# Autodesk Inventor assembly: GCS_AX1
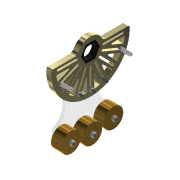
[picture p0: Inventor's stored thumbnail of the model, 180x180]
Saved by Autodesk Inventor 2022 (Build 260153000, 153)
## iProperties
Created: 2022-12-23
Part Number: GCS_AX1
Document SubType Name: Assembly
Designer: alexw
Author: alexw
## Documents named in this file (9)
- C:\Users\alexw\Documents\Inventor\Projects\03_CurrentProjects\MasterThesis\PSM_V1_Rillenkugellager\GCS_AX1.iam
- C:\Users\alexw\Documents\Inventor\Projects\03_CurrentProjects\MasterThesis\PSM_V1_Rillenkugellager\Capstonradialdisc_v2.ipt
- C:\Users\alexw\Documents\Inventor\Projects\03_CurrentProjects\MasterThesis\PSM_V1_Rillenkugellager\CapstonCounterweight_assembly.iam
- C:\Users\alexw\Documents\Inventor\Projects\03_CurrentProjects\MasterThesis\PSM_V1_Rillenkugellager\ContentCenter\de-DE\ISO 10642(1)\ISO 10642 - M6 x  50.ipt
- C:\Users\alexw\Documents\Inventor\Projects\03_CurrentProjects\MasterThesis\PSM_V1_Rillenkugellager\ContentCenter\de-DE\ISO 7093 A\ISO 7093 A - ST 6 - 140 HV.ipt
- C:\Users\alexw\Documents\Inventor\Projects\03_CurrentProjects\MasterThesis\PSM_V1_Rillenkugellager\ContentCenter\de-DE\ISO 4032(2)\ISO 4032 - M6 - ISO.ipt
- C:\Users\alexw\Documents\Inventor\Projects\03_CurrentProjects\MasterThesis\PSM_V1_Rillenkugellager\ContentCenter\de-DE\ISO 4762(2)\ISO 4762 - M6 x 50ISO.ipt
- C:\Users\alexw\Documents\Inventor\Projects\03_CurrentProjects\MasterThesis\PSM_V1_Rillenkugellager\ContentCenter\de-DE\ISO 7092\ISO 7092 - ST 6 - 140 HV.ipt
- C:\Users\alexw\Documents\Inventor\Projects\03_CurrentProjects\MasterThesis\PSM_V1_Rillenkugellager\LS_Cap.ipt
## Components (19 placed, 8 different names)
1. Capstonradialdisc_v2:1
2. CapstonCounterweight_assembly:1 [sub-assembly]
3. ISO 10642 M6x50:1
4. ISO 10642 M6x50:2
5. ISO 10642 M6x50:3
6. ISO 7093 A ST 6 - 140 HV - A:1
7. ISO 7093 A ST 6 - 140 HV - A:2
8. ISO 7093 A ST 6 - 140 HV - A:3
9. ISO 4032 M6:1
10. ISO 4032 M6:2
11. ISO 4762 M6 x 50:1
12. ISO 4762 M6 x 50:2
13. ISO 7092 ST 6 - 140 HV:1
14. ISO 7092 ST 6 - 140 HV:2
15. ISO 7092 ST 6 - 140 HV:3
16. ISO 4032 M6:3
17. ISO 4032 M6:4
18. LS_Cap:1
19. LS_Cap:2
## Relationships (33: Mate 33)
- [Mate]: Capstonradialdisc_v2:1 ↔ CapstonCounterweight_assembly:1
- [Mate]: Capstonradialdisc_v2:1 ↔ CapstonCounterweight_assembly:1
- [Mate]: Capstonradialdisc_v2:1 ↔ CapstonCounterweight_assembly:1
- [Mate]: CapstonCounterweight_assembly:1 ↔ ISO 10642 M6x50:1
- [Mate]: CapstonCounterweight_assembly:1 ↔ ISO 10642 M6x50:2
- [Mate]: CapstonCounterweight_assembly:1 ↔ ISO 10642 M6x50:3
- [Mate]: ISO 10642 M6x50:2 ↔ ISO 7093 A ST 6 - 140 HV - A:1
- [Mate]: Capstonradialdisc_v2:1 ↔ ISO 7093 A ST 6 - 140 HV - A:1
- [Mate]: ISO 10642 M6x50:1 ↔ ISO 7093 A ST 6 - 140 HV - A:2
- [Mate]: Capstonradialdisc_v2:1 ↔ ISO 7093 A ST 6 - 140 HV - A:2
- [Mate]: ISO 10642 M6x50:3 ↔ ISO 7093 A ST 6 - 140 HV - A:3
- [Mate]: Capstonradialdisc_v2:1 ↔ ISO 7093 A ST 6 - 140 HV - A:3
- [Mate]: ISO 10642 M6x50:3 ↔ ISO 4032 M6:1
- [Mate]: ISO 7093 A ST 6 - 140 HV - A:3 ↔ ISO 4032 M6:1
- [Mate]: ISO 10642 M6x50:1 ↔ ISO 4032 M6:2
- [Mate]: ISO 7093 A ST 6 - 140 HV - A:2 ↔ ISO 4032 M6:2
- [Mate]: Capstonradialdisc_v2:1 ↔ ISO 4762 M6 x 50:1
- [Mate]: Capstonradialdisc_v2:1 ↔ ISO 4762 M6 x 50:2
- [Mate]: ISO 4762 M6 x 50:1 ↔ ISO 7092 ST 6 - 140 HV:1
- [Mate]: ISO 4762 M6 x 50:1 ↔ ISO 7092 ST 6 - 140 HV:1
- [Mate]: Capstonradialdisc_v2:1 ↔ ISO 7092 ST 6 - 140 HV:1
- [Mate]: ISO 4762 M6 x 50:2 ↔ ISO 7092 ST 6 - 140 HV:2
- [Mate]: ISO 4762 M6 x 50:2 ↔ ISO 7092 ST 6 - 140 HV:2
- [Mate]: Capstonradialdisc_v2:1 ↔ ISO 7092 ST 6 - 140 HV:2
- [Mate]: ISO 4762 M6 x 50:1 ↔ ISO 7092 ST 6 - 140 HV:3
- [Mate]: Capstonradialdisc_v2:1 ↔ ISO 7092 ST 6 - 140 HV:3
- [Mate]: ISO 4762 M6 x 50:1 ↔ ISO 4032 M6:3
- [Mate]: ISO 7092 ST 6 - 140 HV:3 ↔ ISO 4032 M6:3
- [Mate]: ISO 4762 M6 x 50:2 ↔ ISO 4032 M6:4
- [Mate]: ISO 4762 M6 x 50:1 ↔ LS_Cap:1
- [Mate]: ISO 4032 M6:3 ↔ LS_Cap:1
- [Mate]: ISO 4762 M6 x 50:2 ↔ LS_Cap:2
- [Mate]: ISO 4032 M6:4 ↔ LS_Cap:2
